# Autodesk Inventor assembly: enc-ElectronicsPanel V1 - Assembly
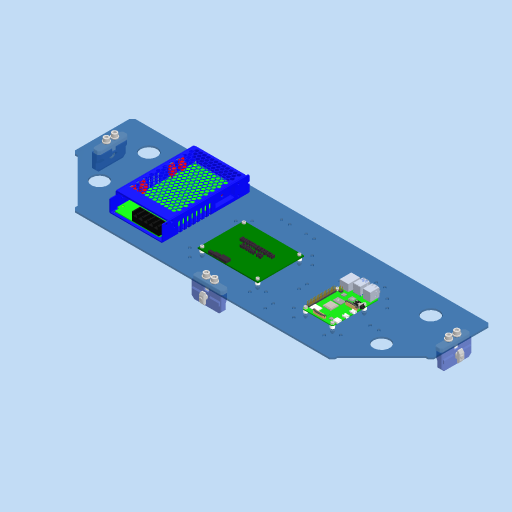
[picture p0: Inventor's stored thumbnail of the model, 512x512]
Saved by Autodesk Inventor 2023.2 (Build 272271000, 271)
## iProperties
Created: 2024-02-16
Part Number: enc-ElectronicsPanel V1 - Assembly
Document SubType Name: Assembly
Designer: Nils Bade
Author: Nils Bade
## Documents named in this file (11)
- C:\Users\nilsb\Documents\Inventor\Projektarbeit-Bade\Enclosure\enc-ElectronicsPanel V1 - Assembly.iam
- C:\Users\nilsb\Documents\Inventor\Projektarbeit-Bade\Enclosure\enc-ElectronicsPanel V1.ipt
- C:\Users\nilsb\Documents\Inventor\Projektarbeit-Bade\Enclosure\Magnet PanelFrame 90deg connected.iam
- C:\Users\nilsb\Documents\Inventor\Projektarbeit-Bade\RatRig_modified\Bigtreetech Skrat V1.ipt
- C:\Users\nilsb\Documents\Inventor\Projektarbeit-Bade\RatRig_modified\MEANWELL RSP-75-24.ipt
- C:\Users\nilsb\Documents\Inventor\Projektarbeit-Bade\RatRig_modified\Raspberry Pi 4\Raspberry Pi 4 Model B\Raspberry Pi 4 Model B.iam
- C:\Users\nilsb\Documents\Inventor\Projektarbeit-Bade\RatRig_modified\Nylon Spacer 3mm X 7mm X 5mm.ipt
- C:\Users\nilsb\Documents\Inventor\Projektarbeit-Bade\Schrauben\Washer Simple M3 - DIN6902.ipt
- C:\Users\nilsb\Documents\Inventor\Projektarbeit-Bade\Schrauben\Cap Head Screw M3x8 v2.ipt
- C:\Users\nilsb\Documents\Inventor\Projektarbeit-Bade\Schrauben\Cap Head Screw M3x16.ipt
- C:\Users\nilsb\Documents\Inventor\Projektarbeit-Bade\RatRig_Standards\Hex Locking Nut - M3 v2.ipt
## Components (43 placed, 10 different names)
1. enc-ElectronicsPanel V1:1 — Passend:1, Passend:2, Passend:3, Passend:4, Passend:5, Passend:6, Passend:7, Passend:8, Passend:9, Passend:10, Winkel:1, Winkel:2, Passend:13, Passend:14, Passend:24, Passend:33, Passend:35, Passend:36, Passend:37, Passend:38, Passend:39, Passend:40, Passend:41, Passend:42, Passend:43, Passend:44, Passend:47, Passend:49, Passend:50, Passend:51, Passend:52, Passend:53, Passend:54, Passend:55, Passend:56, Passend:87, Passend:88
2. Magnet PanelFrame 90deg connected:1 [sub-assembly] — Passend:1, Passend:2, Passend:3
3. Magnet PanelFrame 90deg connected:2 [sub-assembly] — Passend:4, Passend:5, Passend:6
4. Magnet PanelFrame 90deg connected:3 [sub-assembly] — Passend:7, Passend:8, Passend:9
5. MEANWELL RSP-75-24:1 — Passend:10, Winkel:1, Passend:13
6. Washer Simple M3 - DIN6902:2 — Passend:35, Passend:54, Passend:58
7. Washer Simple M3 - DIN6902:6 — Passend:37, Passend:53, Passend:57
8. Cap Head Screw M3x8 v2:1 — Passend:55, Passend:58
9. Cap Head Screw M3x8 v2:2 — Passend:56, Passend:57
10. Bigtreetech Skrat V1:1 — Winkel:2, Passend:14, Passend:16, Passend:17, Passend:18, Passend:19, Passend:20, Passend:21, Passend:22, Passend:23, Passend:71, Passend:72, Passend:73, Passend:74, Passend:79, Passend:80, Passend:81, Passend:82
11. Nylon Spacer 3mm X 7mm X 5mm:1 — Passend:16, Passend:21
12. Nylon Spacer 3mm X 7mm X 5mm:2 — Passend:17, Passend:22
13. Nylon Spacer 3mm X 7mm X 5mm:3 — Passend:18, Passend:23
14. Nylon Spacer 3mm X 7mm X 5mm:4 — Passend:19, Passend:20, Passend:24
15. Washer Simple M3 - DIN6902:1 — Passend:36, Passend:52, Passend:77
16. Washer Simple M3 - DIN6902:3 — Passend:39, Passend:49, Passend:75
17. Washer Simple M3 - DIN6902:5 — Passend:38, Passend:51, Passend:78
18. Washer Simple M3 - DIN6902:10 — Passend:43, Passend:50, Passend:76
19. Cap Head Screw M3x16:1 — Passend:59, Passend:71, Passend:82
20. Cap Head Screw M3x16:2 — Passend:60, Passend:72, Passend:79
21. Cap Head Screw M3x16:3 — Passend:61, Passend:73, Passend:80
22. Cap Head Screw M3x16:4 — Passend:62, Passend:74, Passend:81
23. Hex Locking Nut - M3 v2:1 — Passend:59, Passend:75
24. Hex Locking Nut - M3 v2:2 — Passend:60, Passend:78
25. Hex Locking Nut - M3 v2:3 — Passend:61, Passend:77
26. Hex Locking Nut - M3 v2:4 — Passend:62, Passend:76
27. Raspberry Pi 4 Model B:1 [sub-assembly] — Passend:25, Passend:26, Passend:27, Passend:28, Passend:29, Passend:30, Passend:31, Passend:32, Passend:67, Passend:68, Passend:69, Passend:70, Passend:83, Passend:84, Passend:85, Passend:86
28. Nylon Spacer 3mm X 7mm X 5mm:5 — Passend:25, Passend:29
29. Nylon Spacer 3mm X 7mm X 5mm:6 — Passend:26, Passend:32, Passend:88
30. Nylon Spacer 3mm X 7mm X 5mm:7 — Passend:27, Passend:30
31. Nylon Spacer 3mm X 7mm X 5mm:8 — Passend:28, Passend:31, Passend:33
32. Washer Simple M3 - DIN6902:4 — Passend:42, Passend:91, Passend:95
33. Washer Simple M3 - DIN6902:7 — Passend:40, Passend:47, Passend:94
34. Washer Simple M3 - DIN6902:8 — Passend:41, Passend:90, Passend:92
35. Washer Simple M3 - DIN6902:9 — Passend:44, Passend:89, Passend:93
36. Cap Head Screw M3x16:5 — Passend:63, Passend:67, Passend:83, Passend:91
37. Cap Head Screw M3x16:6 — Passend:64, Passend:68, Passend:84
38. Cap Head Screw M3x16:7 — Passend:65, Passend:69, Passend:85, Passend:89
39. Cap Head Screw M3x16:8 — Passend:66, Passend:70, Passend:86, Passend:87, Passend:90
40. Hex Locking Nut - M3 v2:5 — Passend:63, Passend:95
41. Hex Locking Nut - M3 v2:6 — Passend:64, Passend:94
42. Hex Locking Nut - M3 v2:7 — Passend:65, Passend:93
43. Hex Locking Nut - M3 v2:8 — Passend:66, Passend:92
## Relationships (90: Mate 88, Angle 2)
- Passend:1 [Mate]: enc-ElectronicsPanel V1:1 ↔ Magnet PanelFrame 90deg connected:1
- Passend:2 [Mate]: enc-ElectronicsPanel V1:1 ↔ Magnet PanelFrame 90deg connected:1
- Passend:3 [Mate]: enc-ElectronicsPanel V1:1 ↔ Magnet PanelFrame 90deg connected:1
- Passend:4 [Mate]: enc-ElectronicsPanel V1:1 ↔ Magnet PanelFrame 90deg connected:2
- Passend:5 [Mate]: enc-ElectronicsPanel V1:1 ↔ Magnet PanelFrame 90deg connected:2
- Passend:6 [Mate]: enc-ElectronicsPanel V1:1 ↔ Magnet PanelFrame 90deg connected:2
- Passend:7 [Mate]: enc-ElectronicsPanel V1:1 ↔ Magnet PanelFrame 90deg connected:3
- Passend:8 [Mate]: enc-ElectronicsPanel V1:1 ↔ Magnet PanelFrame 90deg connected:3
- Passend:9 [Mate]: enc-ElectronicsPanel V1:1 ↔ Magnet PanelFrame 90deg connected:3
- Passend:10 [Mate]: enc-ElectronicsPanel V1:1 ↔ MEANWELL RSP-75-24:1
- Winkel:1 [Angle] (90 deg): enc-ElectronicsPanel V1:1 ↔ MEANWELL RSP-75-24:1
- Winkel:2 [Angle] (-90 deg): enc-ElectronicsPanel V1:1 ↔ Bigtreetech Skrat V1:1
- Passend:13 [Mate]: enc-ElectronicsPanel V1:1 ↔ MEANWELL RSP-75-24:1
- Passend:14 [Mate]: enc-ElectronicsPanel V1:1 ↔ Bigtreetech Skrat V1:1
- Passend:16 [Mate]: Bigtreetech Skrat V1:1 ↔ Nylon Spacer 3mm X 7mm X 5mm:1
- Passend:17 [Mate]: Bigtreetech Skrat V1:1 ↔ Nylon Spacer 3mm X 7mm X 5mm:2
- Passend:18 [Mate]: Bigtreetech Skrat V1:1 ↔ Nylon Spacer 3mm X 7mm X 5mm:3
- Passend:19 [Mate]: Bigtreetech Skrat V1:1 ↔ Nylon Spacer 3mm X 7mm X 5mm:4
- Passend:20 [Mate]: Bigtreetech Skrat V1:1 ↔ Nylon Spacer 3mm X 7mm X 5mm:4
- Passend:21 [Mate]: Bigtreetech Skrat V1:1 ↔ Nylon Spacer 3mm X 7mm X 5mm:1
- Passend:22 [Mate]: Bigtreetech Skrat V1:1 ↔ Nylon Spacer 3mm X 7mm X 5mm:2
- Passend:23 [Mate]: Bigtreetech Skrat V1:1 ↔ Nylon Spacer 3mm X 7mm X 5mm:3
- Passend:24 [Mate]: enc-ElectronicsPanel V1:1 ↔ Nylon Spacer 3mm X 7mm X 5mm:4
- Passend:25 [Mate]: Raspberry Pi 4 Model B:1 ↔ Nylon Spacer 3mm X 7mm X 5mm:5
- Passend:26 [Mate]: Raspberry Pi 4 Model B:1 ↔ Nylon Spacer 3mm X 7mm X 5mm:6
- Passend:27 [Mate]: Raspberry Pi 4 Model B:1 ↔ Nylon Spacer 3mm X 7mm X 5mm:7
- Passend:28 [Mate]: Raspberry Pi 4 Model B:1 ↔ Nylon Spacer 3mm X 7mm X 5mm:8
- Passend:29 [Mate]: Raspberry Pi 4 Model B:1 ↔ Nylon Spacer 3mm X 7mm X 5mm:5
- Passend:30 [Mate]: Raspberry Pi 4 Model B:1 ↔ Nylon Spacer 3mm X 7mm X 5mm:7
- Passend:31 [Mate]: Raspberry Pi 4 Model B:1 ↔ Nylon Spacer 3mm X 7mm X 5mm:8
- Passend:32 [Mate]: Raspberry Pi 4 Model B:1 ↔ Nylon Spacer 3mm X 7mm X 5mm:6
- Passend:33 [Mate]: enc-ElectronicsPanel V1:1 ↔ Nylon Spacer 3mm X 7mm X 5mm:8
- Passend:35 [Mate]: enc-ElectronicsPanel V1:1 ↔ Washer Simple M3 - DIN6902:2
- Passend:36 [Mate]: enc-ElectronicsPanel V1:1 ↔ Washer Simple M3 - DIN6902:1
- Passend:37 [Mate]: enc-ElectronicsPanel V1:1 ↔ Washer Simple M3 - DIN6902:6
- Passend:38 [Mate]: enc-ElectronicsPanel V1:1 ↔ Washer Simple M3 - DIN6902:5
- Passend:39 [Mate]: enc-ElectronicsPanel V1:1 ↔ Washer Simple M3 - DIN6902:3
- Passend:40 [Mate]: enc-ElectronicsPanel V1:1 ↔ Washer Simple M3 - DIN6902:7
- Passend:41 [Mate]: enc-ElectronicsPanel V1:1 ↔ Washer Simple M3 - DIN6902:8
- Passend:42 [Mate]: enc-ElectronicsPanel V1:1 ↔ Washer Simple M3 - DIN6902:4
- Passend:43 [Mate]: enc-ElectronicsPanel V1:1 ↔ Washer Simple M3 - DIN6902:10
- Passend:44 [Mate]: enc-ElectronicsPanel V1:1 ↔ Washer Simple M3 - DIN6902:9
- Passend:47 [Mate]: enc-ElectronicsPanel V1:1 ↔ Washer Simple M3 - DIN6902:7
- Passend:49 [Mate]: enc-ElectronicsPanel V1:1 ↔ Washer Simple M3 - DIN6902:3
- Passend:50 [Mate]: enc-ElectronicsPanel V1:1 ↔ Washer Simple M3 - DIN6902:10
- Passend:51 [Mate]: enc-ElectronicsPanel V1:1 ↔ Washer Simple M3 - DIN6902:5
- Passend:52 [Mate]: enc-ElectronicsPanel V1:1 ↔ Washer Simple M3 - DIN6902:1
- Passend:53 [Mate]: enc-ElectronicsPanel V1:1 ↔ Washer Simple M3 - DIN6902:6
- Passend:54 [Mate]: enc-ElectronicsPanel V1:1 ↔ Washer Simple M3 - DIN6902:2
- Passend:55 [Mate]: enc-ElectronicsPanel V1:1 ↔ Cap Head Screw M3x8 v2:1
- Passend:56 [Mate]: enc-ElectronicsPanel V1:1 ↔ Cap Head Screw M3x8 v2:2
- Passend:57 [Mate]: Washer Simple M3 - DIN6902:6 ↔ Cap Head Screw M3x8 v2:2
- Passend:58 [Mate]: Washer Simple M3 - DIN6902:2 ↔ Cap Head Screw M3x8 v2:1
- Passend:59 [Mate]: Cap Head Screw M3x16:1 ↔ Hex Locking Nut - M3 v2:1
- Passend:60 [Mate]: Cap Head Screw M3x16:2 ↔ Hex Locking Nut - M3 v2:2
- Passend:61 [Mate]: Cap Head Screw M3x16:3 ↔ Hex Locking Nut - M3 v2:3
- Passend:62 [Mate]: Cap Head Screw M3x16:4 ↔ Hex Locking Nut - M3 v2:4
- Passend:63 [Mate]: Cap Head Screw M3x16:5 ↔ Hex Locking Nut - M3 v2:5
- Passend:64 [Mate]: Cap Head Screw M3x16:6 ↔ Hex Locking Nut - M3 v2:6
- Passend:65 [Mate]: Cap Head Screw M3x16:7 ↔ Hex Locking Nut - M3 v2:7
- Passend:66 [Mate]: Cap Head Screw M3x16:8 ↔ Hex Locking Nut - M3 v2:8
- Passend:67 [Mate]: Raspberry Pi 4 Model B:1 ↔ Cap Head Screw M3x16:5
- Passend:68 [Mate]: Raspberry Pi 4 Model B:1 ↔ Cap Head Screw M3x16:6
- Passend:69 [Mate]: Raspberry Pi 4 Model B:1 ↔ Cap Head Screw M3x16:7
- Passend:70 [Mate]: Raspberry Pi 4 Model B:1 ↔ Cap Head Screw M3x16:8
- Passend:71 [Mate]: Bigtreetech Skrat V1:1 ↔ Cap Head Screw M3x16:1
- Passend:72 [Mate]: Bigtreetech Skrat V1:1 ↔ Cap Head Screw M3x16:2
- Passend:73 [Mate]: Bigtreetech Skrat V1:1 ↔ Cap Head Screw M3x16:3
- Passend:74 [Mate]: Bigtreetech Skrat V1:1 ↔ Cap Head Screw M3x16:4
- Passend:75 [Mate]: Washer Simple M3 - DIN6902:3 ↔ Hex Locking Nut - M3 v2:1
- Passend:76 [Mate]: Washer Simple M3 - DIN6902:10 ↔ Hex Locking Nut - M3 v2:4
- Passend:77 [Mate]: Washer Simple M3 - DIN6902:1 ↔ Hex Locking Nut - M3 v2:3
- Passend:78 [Mate]: Washer Simple M3 - DIN6902:5 ↔ Hex Locking Nut - M3 v2:2
- Passend:79 [Mate]: Bigtreetech Skrat V1:1 ↔ Cap Head Screw M3x16:2
- Passend:80 [Mate]: Bigtreetech Skrat V1:1 ↔ Cap Head Screw M3x16:3
- Passend:81 [Mate]: Bigtreetech Skrat V1:1 ↔ Cap Head Screw M3x16:4
- Passend:82 [Mate]: Bigtreetech Skrat V1:1 ↔ Cap Head Screw M3x16:1
- Passend:83 [Mate]: Raspberry Pi 4 Model B:1 ↔ Cap Head Screw M3x16:5
- Passend:84 [Mate]: Raspberry Pi 4 Model B:1 ↔ Cap Head Screw M3x16:6
- Passend:85 [Mate]: Raspberry Pi 4 Model B:1 ↔ Cap Head Screw M3x16:7
- Passend:86 [Mate]: Raspberry Pi 4 Model B:1 ↔ Cap Head Screw M3x16:8
- Passend:87 [Mate]: enc-ElectronicsPanel V1:1 ↔ Cap Head Screw M3x16:8
- Passend:88 [Mate]: enc-ElectronicsPanel V1:1 ↔ Nylon Spacer 3mm X 7mm X 5mm:6
- Passend:89 [Mate]: Washer Simple M3 - DIN6902:9 ↔ Cap Head Screw M3x16:7
- Passend:90 [Mate]: Washer Simple M3 - DIN6902:8 ↔ Cap Head Screw M3x16:8
- Passend:91 [Mate]: Washer Simple M3 - DIN6902:4 ↔ Cap Head Screw M3x16:5
- Passend:92 [Mate]: Washer Simple M3 - DIN6902:8 ↔ Hex Locking Nut - M3 v2:8
- Passend:93 [Mate]: Washer Simple M3 - DIN6902:9 ↔ Hex Locking Nut - M3 v2:7
- Passend:94 [Mate]: Washer Simple M3 - DIN6902:7 ↔ Hex Locking Nut - M3 v2:6
- Passend:95 [Mate]: Washer Simple M3 - DIN6902:4 ↔ Hex Locking Nut - M3 v2:5
